# Autodesk Inventor assembly: enix_assembly_v2
(part 2 of 2)
- Mate:634: arm_front_rect:2 ↔ ANSI B18.2.4.2M M3x0,5:4
- Mate:635: AS 1427 H - Metric M3 x 10:4 ↔ ANSI B18.2.4.2M M3x0,5:4
- Mate:636: motor_mount:3 ↔ Emax Rs2205 v1:4
- Mate:637: motor_mount:3 ↔ Emax Rs2205 v1:4
- Mate:638: motor_mount:3 ↔ Emax Rs2205 v1:4
- Mate:639: motor_mount:3 ↔ AS 1427 H - Metric M3 x 5:21
- Mate:640: motor_mount:3 ↔ AS 1427 H - Metric M3 x 5:21
- Mate:641: motor_mount:3 ↔ AS 1427 H - Metric M3 x 5:24
- Mate:642: motor_mount:3 ↔ AS 1427 H - Metric M3 x 5:24
- Mate:643: motor_mount:3 ↔ AS 1427 H - Metric M3 x 5:23
- Mate:644: motor_mount:3 ↔ AS 1427 H - Metric M3 x 5:23
- Mate:645: motor_mount:3 ↔ AS 1427 H - Metric M3 x 5:22
- Mate:646: motor_mount:3 ↔ AS 1427 H - Metric M3 x 5:22
- Mate:647: motor_mount:4 ↔ AS 1427 H - Metric M3 x 5:33
- Mate:648: motor_mount:4 ↔ AS 1427 H - Metric M3 x 5:33
- Mate:649: motor_mount:4 ↔ AS 1427 H - Metric M3 x 5:34
- Mate:650: motor_mount:4 ↔ AS 1427 H - Metric M3 x 5:34
- Mate:651: motor_mount:4 ↔ AS 1427 H - Metric M3 x 5:35
- Mate:652: motor_mount:4 ↔ AS 1427 H - Metric M3 x 5:35
- Mate:653: motor_mount:4 ↔ AS 1427 H - Metric M3 x 5:36
- Mate:654: motor_mount:4 ↔ AS 1427 H - Metric M3 x 5:36
- Mate:655: motor_mount:4 ↔ Emax Rs2205 v1:3
- Mate:656: Emax Rs2205 v1:3 ↔ AS 1427 H - Metric M3 x 5:33
- Mate:657: Emax Rs2205 v1:3 ↔ AS 1427 H - Metric M3 x 5:34
- Mate:658: motor_mount:1 ↔ AS 1427 H - Metric M3 x 5:27
- Mate:659: motor_mount:1 ↔ AS 1427 H - Metric M3 x 5:26
- Mate:660: motor_mount:1 ↔ AS 1427 H - Metric M3 x 5:25
- Mate:661: motor_mount:1 ↔ AS 1427 H - Metric M3 x 5:28
- Mate:662: motor_mount:1 ↔ AS 1427 H - Metric M3 x 5:27
- Mate:663: motor_mount:1 ↔ AS 1427 H - Metric M3 x 5:26
- Mate:664: motor_mount:1 ↔ AS 1427 H - Metric M3 x 5:25
- Mate:665: motor_mount:1 ↔ AS 1427 H - Metric M3 x 5:28
- Mate:666: motor_mount:1 ↔ Emax Rs2205 v1:2
- Mate:667: Emax Rs2205 v1:2 ↔ AS 1427 H - Metric M3 x 5:26
- Mate:668: Emax Rs2205 v1:2 ↔ AS 1427 H - Metric M3 x 5:27
- Mate:669: motor_mount:2 ↔ AS 1427 H - Metric M3 x 5:31
- Mate:670: motor_mount:2 ↔ AS 1427 H - Metric M3 x 5:32
- Mate:671: motor_mount:2 ↔ AS 1427 H - Metric M3 x 5:29
- Mate:672: motor_mount:2 ↔ AS 1427 H - Metric M3 x 5:30
- Mate:673: motor_mount:2 ↔ AS 1427 H - Metric M3 x 5:30
- Mate:674: motor_mount:2 ↔ AS 1427 H - Metric M3 x 5:31
- Mate:675: motor_mount:2 ↔ AS 1427 H - Metric M3 x 5:29
- Mate:676: motor_mount:2 ↔ AS 1427 H - Metric M3 x 5:32
- Mate:677: motor_mount:2 ↔ Emax Rs2205 v1:1
- Mate:678: Emax Rs2205 v1:1 ↔ AS 1427 H - Metric M3 x 5:32
- Mate:679: Emax Rs2205 v1:1 ↔ AS 1427 H - Metric M3 x 5:29
- Mate:680: top_plate:1 ↔ AS 1427 H - Metric M2 x 8:55
- Mate:681: top_plate:1 ↔ AS 1427 H - Metric M2 x 8:57
- Mate:682: top_plate:1 ↔ AS 1427 H - Metric M2 x 8:56
- Mate:683: top_plate:1 ↔ AS 1427 H - Metric M2 x 8:59
- Mate:684: arm_socket_l:1 ↔ AS 1427 H - Metric M2 x 8:58
- Mate:685: arm_socket_l:1 ↔ AS 1427 H - Metric M2 x 8:60
- Mate:686: arm_socket_l:2 ↔ AS 1427 H - Metric M2 x 8:62
- Mate:687: arm_socket_l:2 ↔ AS 1427 H - Metric M2 x 8:61
- Mate:688: arm_socket_l:2 ↔ AS 1427 H - Metric M2 x 8:61
- Mate:689: arm_socket_l:2 ↔ AS 1427 H - Metric M2 x 8:62
- Mate:690: top_plate:1 ↔ AS 1427 H - Metric M2 x 8:55
- Mate:691: top_plate:1 ↔ AS 1427 H - Metric M2 x 8:57
- Mate:692: top_plate:1 ↔ AS 1427 H - Metric M2 x 8:69
- Mate:693: top_plate:1 ↔ AS 1427 H - Metric M2 x 8:70
- Mate:694: arm_socket_r:2 ↔ AS 1427 H - Metric M2 x 8:68
- Mate:695: arm_socket_r:2 ↔ AS 1427 H - Metric M2 x 8:67
- Mate:696: top_plate:1 ↔ AS 1427 H - Metric M2 x 8:66
- Mate:697: top_plate:1 ↔ AS 1427 H - Metric M2 x 8:65
- Mate:698: arm_socket_r:1 ↔ AS 1427 H - Metric M2 x 8:64
- Mate:699: arm_socket_r:1 ↔ AS 1427 H - Metric M2 x 8:63
- Mate:700: arm_socket_r:1 ↔ AS 1427 H - Metric M2 x 8:64
- Mate:701: top_plate:1 ↔ AS 1427 H - Metric M2 x 8:66
- Mate:702: top_plate:1 ↔ AS 1427 H - Metric M2 x 8:65
- Mate:703: arm_socket_r:1 ↔ AS 1427 H - Metric M2 x 8:63
- Mate:704: top_plate:1 ↔ AS 1427 H - Metric M2 x 8:59
- Mate:705: top_plate:1 ↔ AS 1427 H - Metric M2 x 8:56
- Mate:706: arm_socket_l:1 ↔ AS 1427 H - Metric M2 x 8:58
- Mate:707: arm_socket_l:1 ↔ AS 1427 H - Metric M2 x 8:60
- Mate:708: top_plate:1 ↔ AS 1427 H - Metric M2 x 8:70
- Mate:709: top_plate:1 ↔ AS 1427 H - Metric M2 x 8:69
- Mate:710: arm_socket_r:2 ↔ AS 1427 H - Metric M2 x 8:68
- Mate:711: arm_socket_r:2 ↔ AS 1427 H - Metric M2 x 8:67
- Mate:712: baseplate:1 ↔ AS 1112 (2) - Metric M2  Type 5:66
- Mate:713: baseplate:1 ↔ AS 1112 (2) - Metric M2  Type 5:65
- Mate:714: AS 1427 H - Metric M2 x 8:63 ↔ AS 1112 (2) - Metric M2  Type 5:65
- Mate:715: AS 1427 H - Metric M2 x 8:64 ↔ AS 1112 (2) - Metric M2  Type 5:66
- Mate:716: arm_socket_r:1 ↔ AS 1112 (2) - Metric M2  Type 5:64
- Mate:717: AS 1427 H - Metric M2 x 8:66 ↔ AS 1112 (2) - Metric M2  Type 5:64
- Mate:718: arm_socket_r:1 ↔ AS 1112 (2) - Metric M2  Type 5:63
- Mate:719: AS 1427 H - Metric M2 x 8:65 ↔ AS 1112 (2) - Metric M2  Type 5:63
- Mate:720: arm_socket_r:2 ↔ AS 1112 (2) - Metric M2  Type 5:67
- Mate:721: AS 1427 H - Metric M2 x 8:69 ↔ AS 1112 (2) - Metric M2  Type 5:67
- Mate:722: arm_socket_r:2 ↔ AS 1112 (2) - Metric M2  Type 5:70
- Mate:723: AS 1427 H - Metric M2 x 8:70 ↔ AS 1112 (2) - Metric M2  Type 5:70
- Mate:724: baseplate:1 ↔ AS 1112 (2) - Metric M2  Type 5:69
- Mate:725: baseplate:1 ↔ AS 1112 (2) - Metric M2  Type 5:68
- Mate:726: AS 1427 H - Metric M2 x 8:67 ↔ AS 1112 (2) - Metric M2  Type 5:68
- Mate:727: AS 1427 H - Metric M2 x 8:68 ↔ AS 1112 (2) - Metric M2  Type 5:69
- Mate:728: arm_socket_l:1 ↔ AS 1112 (2) - Metric M2  Type 5:77
- Mate:729: AS 1427 H - Metric M2 x 8:56 ↔ AS 1112 (2) - Metric M2  Type 5:77
- Mate:730: arm_socket_l:1 ↔ AS 1112 (2) - Metric M2  Type 5:75
- Mate:731: AS 1427 H - Metric M2 x 8:59 ↔ AS 1112 (2) - Metric M2  Type 5:75
- Mate:732: baseplate:1 ↔ AS 1112 (2) - Metric M2  Type 5:78
- Mate:733: baseplate:1 ↔ AS 1112 (2) - Metric M2  Type 5:76
- Mate:734: AS 1427 H - Metric M2 x 8:60 ↔ AS 1112 (2) - Metric M2  Type 5:76
- Mate:735: AS 1427 H - Metric M2 x 8:58 ↔ AS 1112 (2) - Metric M2  Type 5:78
- Mate:736: arm_socket_l:2 ↔ AS 1112 (2) - Metric M2  Type 5:71
- Mate:737: AS 1427 H - Metric M2 x 8:55 ↔ AS 1112 (2) - Metric M2  Type 5:71
- Mate:738: baseplate:1 ↔ AS 1112 (2) - Metric M2  Type 5:72
- Mate:739: AS 1427 H - Metric M2 x 8:62 ↔ AS 1112 (2) - Metric M2  Type 5:72
- Mate:740: baseplate:1 ↔ AS 1112 (2) - Metric M2  Type 5:74
- Mate:741: AS 1427 H - Metric M2 x 8:61 ↔ AS 1112 (2) - Metric M2  Type 5:74
- Mate:742: arm_socket_l:2 ↔ AS 1112 (2) - Metric M2  Type 5:73
- Mate:743: AS 1427 H - Metric M2 x 8:57 ↔ AS 1112 (2) - Metric M2  Type 5:73
- Mate:744: top_plate:1 ↔ AS 1427 H - Metric M3 x 30:1
- Mate:745: top_plate:1 ↔ AS 1427 H - Metric M3 x 30:1
- Mate:746: top_plate:1 ↔ AS 1427 H - Metric M3 x 30:2
- Mate:747: top_plate:1 ↔ AS 1427 H - Metric M3 x 30:4
- Mate:748: top_plate:1 ↔ AS 1427 H - Metric M3 x 30:3
- Mate:749: top_plate:1 ↔ AS 1427 H - Metric M3 x 30:3
- Mate:750: top_plate:1 ↔ AS 1427 H - Metric M3 x 30:4
- Mate:751: top_plate:1 ↔ AS 1427 H - Metric M3 x 30:2
- Mate:752: baseplate:1 ↔ ANSI B18.2.4.2M M3x0,5:8
- Mate:753: baseplate:1 ↔ ANSI B18.2.4.2M M3x0,5:6
- Mate:754: AS 1427 H - Metric M3 x 30:2 ↔ ANSI B18.2.4.2M M3x0,5:6
- Mate:755: AS 1427 H - Metric M3 x 30:1 ↔ ANSI B18.2.4.2M M3x0,5:8
- Mate:756: baseplate:1 ↔ ANSI B18.2.4.2M M3x0,5:5
- Mate:757: baseplate:1 ↔ ANSI B18.2.4.2M M3x0,5:5
- Mate:758: baseplate:1 ↔ ANSI B18.2.4.2M M3x0,5:7
- Mate:759: AS 1427 H - Metric M3 x 30:4 ↔ ANSI B18.2.4.2M M3x0,5:7
- Mate:795: baseplate:1 ↔ transformer_mount_new:1
- Mate:796: baseplate:1 ↔ transformer_mount_new:1
- Mate:797: baseplate:1 ↔ transformer_mount_new:1
- Mate:798: transformer:2 ↔ transformer_mount_new:1
- Mate:799: transformer:2 ↔ transformer_mount_new:1
- Mate:800: transformer:2 ↔ transformer_mount_new:1
- Mate:801: transformer_mount_new:1 ↔ AS 1427 H - Metric M2 x 8:77
- Mate:802: transformer_mount_new:1 ↔ AS 1427 H - Metric M2 x 8:77
- Mate:803: transformer_mount_new:1 ↔ AS 1427 H - Metric M2 x 8:78
- Mate:804: transformer_mount_new:1 ↔ AS 1427 H - Metric M2 x 8:78
- Mate:805: baseplate:1 ↔ AS 1112 (2) - Metric M2  Type 5:85
- Mate:806: AS 1427 H - Metric M2 x 8:77 ↔ AS 1112 (2) - Metric M2  Type 5:85
- Mate:807: baseplate:1 ↔ AS 1112 (2) - Metric M2  Type 5:86
- Mate:808: AS 1427 H - Metric M2 x 8:78 ↔ AS 1112 (2) - Metric M2  Type 5:86
- Mate:809: transformer:2 ↔ AS 1427 H - Metric M2 x 8:79
- Mate:810: transformer:2 ↔ AS 1427 H - Metric M2 x 8:79
- Mate:811: transformer:2 ↔ AS 1427 H - Metric M2 x 8:80
- Mate:812: transformer:2 ↔ AS 1427 H - Metric M2 x 8:80
- Mate:813: transformer_mount_new:1 ↔ AS 1112 (2) - Metric M2  Type 5:87
- Mate:814: AS 1427 H - Metric M2 x 8:79 ↔ AS 1112 (2) - Metric M2  Type 5:87
- Mate:815: transformer_mount_new:1 ↔ AS 1112 (2) - Metric M2  Type 5:88
- Mate:816: AS 1427 H - Metric M2 x 8:80 ↔ AS 1112 (2) - Metric M2  Type 5:88
- Mate:817: baseplate:1 ↔ transformer_mount_new:2
- Mate:818: baseplate:1 ↔ transformer_mount_new:2
- Mate:819: baseplate:1 ↔ transformer_mount_new:2
- Mate:820: transformer_mount_new:2 ↔ transformer:3
- Mate:821: transformer_mount_new:2 ↔ transformer:3
- Mate:822: transformer_mount_new:2 ↔ transformer:3
- [Mate]: AS 1427 H - Metric M2 x 8:81 ↔ AS 1112 (2) - Metric M2  Type 5:89
- [Mate]: AS 1427 H - Metric M2 x 8:82 ↔ AS 1112 (2) - Metric M2  Type 5:90
- Mate:825: transformer_mount_new:2 ↔ AS 1427 H - Metric M2 x 8:81
- Mate:826: transformer_mount_new:2 ↔ AS 1427 H - Metric M2 x 8:81
- Mate:827: baseplate:1 ↔ AS 1112 (2) - Metric M2  Type 5:89
- Mate:828: transformer_mount_new:2 ↔ AS 1427 H - Metric M2 x 8:82
- Mate:829: transformer_mount_new:2 ↔ AS 1427 H - Metric M2 x 8:82
- Mate:830: baseplate:1 ↔ AS 1112 (2) - Metric M2  Type 5:90
- Mate:831: transformer:3 ↔ AS 1427 H - Metric M2 x 8:83
- Mate:832: transformer:3 ↔ AS 1427 H - Metric M2 x 8:83
- Mate:833: transformer:3 ↔ AS 1427 H - Metric M2 x 8:84
- Mate:834: transformer:3 ↔ AS 1427 H - Metric M2 x 8:84
- Mate:835: transformer_mount_new:2 ↔ AS 1112 (2) - Metric M2  Type 5:91
- Mate:836: AS 1427 H - Metric M2 x 8:84 ↔ AS 1112 (2) - Metric M2  Type 5:91
- Mate:837: transformer_mount_new:2 ↔ AS 1112 (2) - Metric M2  Type 5:92
- Mate:838: AS 1427 H - Metric M2 x 8:83 ↔ AS 1112 (2) - Metric M2  Type 5:92
- Mate:839: cam_holder:1 ↔ kamera:1
- Mate:840: cam_holder:1 ↔ kamera:1
- Mate:841: cam_holder:1 ↔ kamera:1
- Mate:842: kamera:1 ↔ AS 1427 H - Metric M2 x 8:85
- Mate:844: kamera:1 ↔ AS 1427 H - Metric M2 x 8:87
- Mate:845: kamera:1 ↔ AS 1427 H - Metric M2 x 8:86
- Mate:846: kamera:1 ↔ AS 1427 H - Metric M2 x 8:88
- Mate:847: kamera:1 ↔ AS 1427 H - Metric M2 x 8:87
- Mate:848: kamera:1 ↔ AS 1427 H - Metric M2 x 8:88
- Mate:849: kamera:1 ↔ AS 1427 H - Metric M2 x 8:86
- Mate:850: kamera:1 ↔ AS 1427 H - Metric M2 x 8:85
- Mate:851: AS 1112 (2) - Metric M2  Type 5:31 ↔ AS 1427 H - Metric M2 x 8:86
- Mate:852: AS 1112 (2) - Metric M2  Type 5:29 ↔ AS 1427 H - Metric M2 x 8:88
## Named parameters: sa_0 = -13.8611, sa_1 = 0, sa_2 = 999.904, sa_3 = -5.52663, sa_4 = 0, sa_5 = 999.985, sa_6 = 0, sa_7 = -500, sa_8 = -0, d930_d913 = 0 mm, d931_d913 = 0 mm
note: some values were not read from the file. Shown as the stored number, unit unknown: "sa_0", "sa_1", "sa_2", "sa_3", "sa_4", "sa_5", "sa_6", "sa_7", "sa_8".
